# Autodesk Inventor assembly: MotorFufuPounder
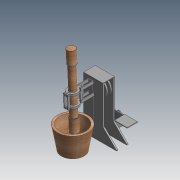
[picture p0: Inventor's stored thumbnail of the model, 180x180]
Saved by Autodesk Inventor 2015 (Build 190159000, 159)
## iProperties
Created: 2014-08-31
Part Number: MotorFufuPounder
Document SubType Name: Assembly
Designer: shohei
Author: shohei
## Documents named in this file (3)
- C:\Users\shohei\Documents\Inventor\FufuPounder\MotorFufuPounder.iam
- C:\Users\shohei\Documents\Inventor\FufuPounder\rev6.iam
- C:\Users\shohei\Documents\Inventor\FufuPounderLeverType\GearAssembly_rev1.iam
## Components (2 placed, 2 different names)
1. rev6:1 [sub-assembly] — Flush:1
2. GearAssembly_rev1:1 [sub-assembly] — Flush:1
## Relationships (1: Flush 1)
- Flush:1: rev6:1 ↔ GearAssembly_rev1:1
